# Autodesk Inventor assembly: Friction Wheel Assembly dtp2.0
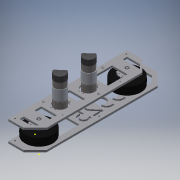
[picture p0: Inventor's stored thumbnail of the model, 180x180]
Saved by Autodesk Inventor 2017 (Build 210142000, 142)
## iProperties
Created: 2017-08-09
Part Number: Friction Wheel Assembly dtp2.0
Document SubType Name: Assembly
Designer: User
Author: User
## Documents named in this file (5)
- C:\Robotics\CAD\2016-17_CAD\Friction Wheel Assembly dtp2.0.iam
- C:\Robotics\CAD\2016-17_CAD\DriveTrain\DrainTrainPlate2.0LeftOutside.iam
- C:\Robotics\CAD\2016-17_CAD\DriveTrain\DriveTrainPlate2.0LeftInside.ipt
- C:\Robotics\CAD\2016-17_CAD\DriveTrain\wheel sub assembly traction wheels.iam
- C:\Robotics\CAD\2016-17_CAD\DriveTrain\motor sub assembley.iam
## Components (6 placed, 4 different names)
1. DrainTrainPlate2.0LeftOutside:1 [sub-assembly] — Mate:3, Mate:4, Mate:7
2. DriveTrainPlate2.0LeftInside:1 — Mate:1, Mate:2, Mate:5, Mate:6, Mate:8, Mate:9
3. wheel sub assembly traction wheels:1 [sub-assembly] — Mate:5, Mate:6, Mate:7, Flush:1
4. wheel sub assembly traction wheels:2 [sub-assembly] — Mate:1, Mate:2, Mate:3, Mate:4, Flush:2
5. motor sub assembley:3 [sub-assembly] — Mate:8, Flush:1
6. motor sub assembley:4 [sub-assembly] — Mate:9, Flush:2
## Relationships (11: Mate 9, Flush 2)
- Mate:1 (6.35 mm): DriveTrainPlate2.0LeftInside:1 ↔ wheel sub assembly traction wheels:2
- Mate:2: DriveTrainPlate2.0LeftInside:1 ↔ wheel sub assembly traction wheels:2
- Mate:3: DrainTrainPlate2.0LeftOutside:1 ↔ wheel sub assembly traction wheels:2
- Mate:4 (3.175 mm): DrainTrainPlate2.0LeftOutside:1 ↔ wheel sub assembly traction wheels:2
- Mate:5 (6.35 mm): DriveTrainPlate2.0LeftInside:1 ↔ wheel sub assembly traction wheels:1
- Mate:6: DriveTrainPlate2.0LeftInside:1 ↔ wheel sub assembly traction wheels:1
- Mate:7: DrainTrainPlate2.0LeftOutside:1 ↔ wheel sub assembly traction wheels:1
- Mate:8: DriveTrainPlate2.0LeftInside:1 ↔ motor sub assembley:3
- Flush:1: wheel sub assembly traction wheels:1 ↔ motor sub assembley:3
- Mate:9: DriveTrainPlate2.0LeftInside:1 ↔ motor sub assembley:4
- Flush:2: wheel sub assembly traction wheels:2 ↔ motor sub assembley:4
